# Autodesk Inventor assembly: GPA32GT2060-A-P10
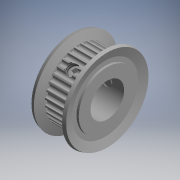
[picture p0: Inventor's stored thumbnail of the model, 180x180]
Saved by Autodesk Inventor 2017.3 (Build 213256000, 256)
## iProperties
Category: PARTsolutions
Company: MISUMI
Part Number: GPA32GT2060-A-P10
Catalog Web Link: www.cadenas.de
Description: GPA__GT2040, GPA__GT2060, GPA__GT2090-High Torque Timing Pulleys 2GT Type
Vendor: MISUMI
Document SubType Name: Assembly
Designer: partserver
Manufacturer: MISUMI
Mass: 2.42658 g
Surface Area: 25.5873 cm^2
Volume: 2.42658 cm^3
Density: 1 g/cm^3
Title: GPA32GT2060-A-P10
Author: Cadenas PARTsolutions
Comments: High Torque Timing Pulleys 2GT Type
PSOL_IDENT_0: {$CADENAS_DATA\23d-libs\misumi\metric\51_timing_pulleys\gpa_gt2_asmtab.prj},392 {VTYP=3D},{STYP=ASST
PSOL_IDENT_1: AB},{NB=GPA32GT2060-A-P10},{LINA=GPA32GT2060-A-P10},{NN=GPA__GT2040, GPA__GT2060, GPA__GT2090},{DATE=
PSOL_IDENT_2: 09.09.2019 15:28:20},{GEOMDATE=17.12.2018 08:25:58},{VERSION=},{LINEID=120},{WBVAR=TNW,PS,SBS,DD,Z,J
PSOL_IDENT_3: ,Q,R,S,T,ALT1,ALT2,M,QSC,QFC,QTC,ALT3,K,KSC,KFC,KTC,ALT4,ZM,ZSC,ZFC,ZTC,ALT5,BC,ALT6,ALT7,ALT8,FC},{
PSOL_IDENT_4: WBNUMERIC=DD,Z,J,Q,R,S,T,QSC,QFC,QTC,K,KSC,KFC,KTC,ZSC,ZFC,ZTC,BC,FC}  {NB=GPA32GT2060-A-P10},{LINA=
PSOL_IDENT_5: GPA32GT2060-A-P10},{KT=DUMMY},{PN=GPA32GT2060-A-P10},{TYPE=GPA},{NT=32},{TNW=GT2060},{BW=6},{A=7.0},
PSOL_IDENT_6: {W=10.3},{L=18.0},{PS=A},{PSA= 'A','B' },{SBS=P},{SBSALG= 'H','Round Hole','P','Round Hole+Tap','V','
PSOL_IDENT_7: Stepped Hole','Y','Both Ends Stepped Hole' },{DD=10.00},{DDALG=[5:6/1],[6.35],[7:10/1]},{DDHA=[5:6/1
PSOL_IDENT_8: ],[6.35],[7:13/1]},{DDHB=[5:6/1],[6.35],[7:9/1]},{DDPA=[5:6/1],[6.35],[7:10/1]},{DDPB=[5:6/1]},{DDNA=
PSOL_IDENT_9: },{DDNB=},{DDNKA=0},{DDNKB=0},{DDVA=[5:6/1],[6.35],[7:11/1]},{DDVFB=[5:6/1],[6.35],[7:7/1]},{DDYA=[5
PSOL_IDENT_10: :11/1]},{Z=0},{ZALG=0},{ZMIN=12},{ZAMAX=13},{ZBMAX=9},{J=0.0},{JALG=0},{JMAX=8.3},{Q=0},{R=0},{QRALG=
PSOL_IDENT_11: 0},{QRMIN=12},{QRMAX=13},{S=0.0},{SALG=0},{SMAX=4.300},{T=0.0},{TALG=0},{TMAX=5.000},{PD=20.37},{OD=
PSOL_IDENT_12: 19.86},{D=13},{DE=17},{DDZ=10},{F=25},{E=17},{BB=0},{TT=0},{M1=4},{AC=M4x3},{ALT1=},{ALT1A= '','w/o
PSOL_IDENT_13: Set Screw Angle','-KC90','with KC90 (Set Screw Angle)' },{ANG=123.75},{ALT2=},{ALT2A= '','Not applic
PSOL_IDENT_14: able' },{M=N/A},{MALG= 'N/A' },{MM=0.000},{MPHD=0.000},{MA= 'N/A' },{MSA= 'N/A' },{QSC=0.0},{QSCA=0}
PSOL_IDENT_15: ,{QFC=0.0},{QFCA=0},{QTC=0.0},{QTCA=0},{QPCDMIN=14},{QPCDMINALG=14},{QPCDMAX=13},{ALT2PN=},{ALT3=},{
PSOL_IDENT_16: ALT3A= '','Not applicable' },{K=0.0},{KA=0},{KAMIN=4},{KAMAX=0},{KSMAX=0},{KSC=0.0},{KSCA=0},{KFC=0.
PSOL_IDENT_17: 0},{KFCA=0},{KTC=0.0},{KTCA=0},{KSCMIN=14.000},{KPCDMIN=14.000},{KPCDMINALG=18.000},{KPCDMAX=13.000}
PSOL_IDENT_18: ,{ALT3PN=},{ALT4=},{ALT4ALG= '','Not applicable' },{ALT4MIN=20.500},{ALT4MAX=6.500},{ZM=N/A},{ZMALG=
PSOL_IDENT_19: 'N/A' },{ZMFTALG= 'N/A' },{ZMSALG= 'N/A' },{ZMDD1=0.0},{ZMDD2=0.0},{ZMHH=0.0},{ZSC=0.0},{ZSCALG=[0]
PSOL_IDENT_20: },{ZFC=0.0},{ZFCALG=[0]},{ZTC=0.0},{ZTCALG=[0]},{ZPCDMIN=0.000},{ZPCDMINALG=0.000},{ZPCDMAX=13.000},
PSOL_IDENT_21: {ALT4PN=},{ALT5=},{ALT5ALG= '','Not applicable' },{ALT5PN=},{BC=0.0},{BCALG=0},{BCMIN=7.000},{BCMAX=
PSOL_IDENT_22: 7.700},{ALT6=},{ALT7=},{ALT7ALG= '','w/o Flange Attached on One Side Only','-RFC','with RFC (Flange
PSOL_IDENT_23: Attached on The Boss Side Only)','-LFC','with LFC (Flange Attached on The Opposite Side Only)' },{AL
PSOL_IDENT_24: T8=},{ALT8ALG='','w/o FC (Flange Cut)','-FC','with FC (Flange Cut)'},{ALT8PN=},{FC=0.0},{FCA=0},{ODA
PSOL_IDENT_25: INT=23.000},{FCMIN=21},{FCMAX=23},{WLBC=10.3},{SL=5},{SL2=5},{KTT=5},{KYY=4.93},{TAP=0},{PPATH=gpa__
PSOL_IDENT_26: gt2/gpa_gt2_asmtpl.prj}
NB: GPA32GT2060-A-P10
NN: GPA__GT2040, GPA__GT2060, GPA__GT2090
NT: 32
NBSYN: $PN.
LINA: GPA32GT2060-A-P10
CATALOG: Misumi
PN: GPA32GT2060-A-P10
TNW: GT2060
A: 7
W: 10.3
L: 18
PS: A
SBS: Round Hole+Tap
DD: 10
Z: 0
J: 0
Q: 0
R: 0
S: 0
T: 0
PD: 20.37
OD: 19.86
D: 13
F: 25
E: 17
AC: M4x3
ALT1: w/o Set Screw Angle
ALT2: Not applicable
M: N/A
QSC: 0
QFC: 0
QTC: 0
ALT3: Not applicable
K: 0
KSC: 0
KFC: 0
KTC: 0
ALT4: Not applicable
ZM: N/A
ZMDD1: 0
ZMDD2: 0
ZMHH: 0
ZSC: 0
ZFC: 0
ZTC: 0
ALT5: Not applicable
BC: 0
ALT6: w/o Flange not Attached
ALT7: w/o Flange Attached on One Side Only
ALT8: w/o FC (Flange Cut)
FC: 0
SUPPLIER: MISUMI
ARTICLENO: GPA32GT2060-A-P10
BOMINFO: GPA32GT2060-A-P10
CREATOR: CADENAS GmbH
## Documents named in this file (3)
- e:\temp\worker_21\temp\exporttempdir_2604_328_Ao9X5\format_0\GPA32GT2060-A-P10.iam
- e:\temp\worker_21\temp\exporttempdir_2604_328_Ao9X5\format_0\GPA32GT2060-A-P10_b.ipt
- e:\temp\worker_21\temp\exporttempdir_2604_328_Ao9X5\format_0\SET-SCREW4-3.ipt
## Components (3 placed, 2 different names)
1. GPA32GT2060-A-P10_b:1 — to_Screw_A1_Z@1 <-> CP_Z@2, to_Screw_A2_XY@1 <-> CP_XY@3, to_Screw_A2_Z@1 <-> CP_Z@3, to_Screw_A2_YZ@1 <-> CP_YZ@3
2. SET-SCREW4-3:1 — to_Screw_A1_Z@1 <-> CP_Z@2
3. SET-SCREW4-3:2 — to_Screw_A2_XY@1 <-> CP_XY@3, to_Screw_A2_Z@1 <-> CP_Z@3, to_Screw_A2_YZ@1 <-> CP_YZ@3
## Relationships (4: Mate 3, Angle 1)
- to_Screw_A1_Z@1 <-> CP_Z@2 [Mate]: GPA32GT2060-A-P10_b:1 ↔ SET-SCREW4-3:1
- to_Screw_A2_XY@1 <-> CP_XY@3 [Mate]: GPA32GT2060-A-P10_b:1 ↔ SET-SCREW4-3:2
- to_Screw_A2_Z@1 <-> CP_Z@3 [Mate]: GPA32GT2060-A-P10_b:1 ↔ SET-SCREW4-3:2
- to_Screw_A2_YZ@1 <-> CP_YZ@3 [Angle] (0 deg): GPA32GT2060-A-P10_b:1 ↔ SET-SCREW4-3:2
